# Autodesk Inventor assembly: ExtruderSatoer
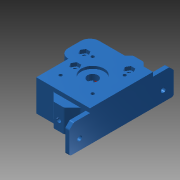
[picture p0: Inventor's stored thumbnail of the model, 180x180]
Saved by Autodesk Inventor 2015 SP1 (Build 190203100, 203)
## iProperties
Created: 2015-05-03
Part Number: ExtruderSatoer
Document SubType Name: Assembly
Designer: Jack
Author: Jack
## Documents named in this file (3)
- C:\Users\Jack\ownCloud\Projects\CrossBot\InventorModel\Extruder\ExtruderSatoer\ExtruderSatoer.iam
- C:\Users\Jack\ownCloud\Projects\CrossBot\InventorModel\Extruder\ExtruderSatoer\ExtruderSatoerBody.ipt
- C:\Users\Jack\ownCloud\Projects\CrossBot\InventorModel\Extruder\ExtruderSatoer\ExtruderSatoerMotorMount.ipt
## Components (2 placed, 2 different names)
1. ExtruderSatoerBody:1 — Mate:7, Mate:8, Mate:9
2. ExtruderSatoerMotorMount:1 — Mate:7, Mate:8, Mate:9
## Relationships (3: Mate 3)
- Mate:7 (0.25 mm): ExtruderSatoerBody:1 ↔ ExtruderSatoerMotorMount:1
- Mate:8 (0.25 mm): ExtruderSatoerBody:1 ↔ ExtruderSatoerMotorMount:1
- Mate:9: ExtruderSatoerBody:1 ↔ ExtruderSatoerMotorMount:1
